# Autodesk Inventor assembly: Convery Digital Prototype
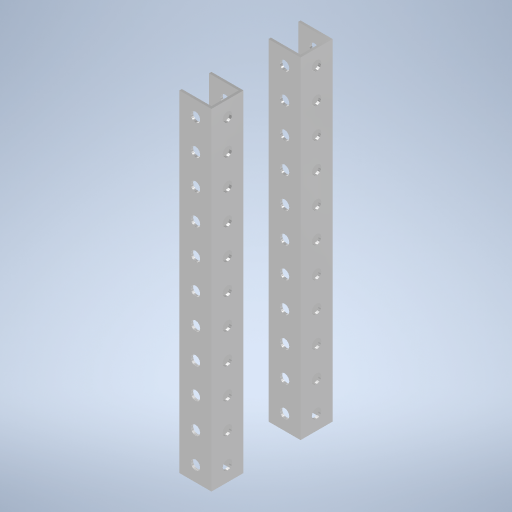
[picture p0: Inventor's stored thumbnail of the model, 512x512]
Saved by Autodesk Inventor 2024 (Build 280153020, 153B)
## iProperties
Created: 2024-02-06
Part Number: Convery Digital Prototype
Document SubType Name: Assembly
Designer: scottst
Author: scottst
## Documents named in this file (2)
- H:\Robotics Club\3D Models\Mr Scott\Convery Digital Prototype.iam
- H:\Robotics Club\3D Models\Mr Scott\C-Channel 11in.ipt
## Components (2 placed, 1 different names)
1. C-Channel 11in:1 — Flush:1, Flush:2
2. C-Channel 11in:2 — Flush:1, Flush:2
## Relationships (2: Flush 2)
- Flush:1: C-Channel 11in:1 ↔ C-Channel 11in:2
- Flush:2: C-Channel 11in:1 ↔ C-Channel 11in:2
